# Autodesk Inventor assembly: Craftsman Socket U-Joint
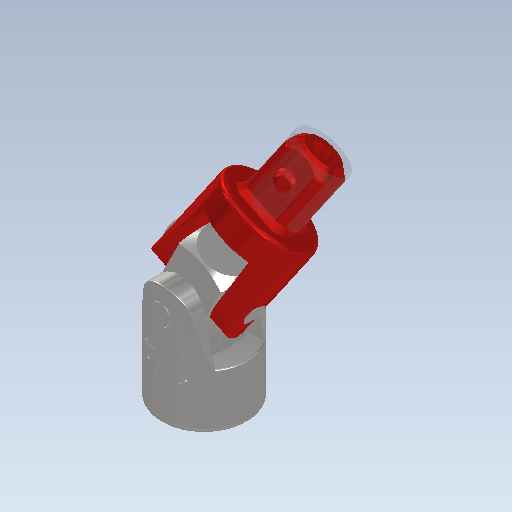
[picture p0: Inventor's stored thumbnail of the model, 512x512]
Saved by Autodesk Inventor 2020 (Build 240168000, 168)
## iProperties
Created: 2013-08-30
Part Number: Craftsman Socket U-Joint
Document SubType Name: Assembly
Designer: Vikki
Sending System: SolidWorks 2012
Last Author: MBryant
Last Saved: 2013-08-30
WEIGHT: 0.048
MX_MODIFIED: true
Author: Vikki
## Documents named in this file (4)
- D:\borewell rescuebot\pll manipulator files\sps manipulator\craftsman-3-pc-universal-joint-set-1.snapshot.1\Craftsman Socket U-Joint.iam
- D:\borewell rescuebot\pll manipulator files\sps manipulator\craftsman-3-pc-universal-joint-set-1.snapshot.1\Craftsman Socket U-Joint Base.ipt
- D:\borewell rescuebot\pll manipulator files\sps manipulator\craftsman-3-pc-universal-joint-set-1.snapshot.1\Craftsman Socket U-Joint Intermediate Body.ipt
- D:\borewell rescuebot\pll manipulator files\sps manipulator\craftsman-3-pc-universal-joint-set-1.snapshot.1\Craftsman Socket U-Joint Drive.ipt
## Components (3 placed, 3 different names)
1. Craftsman Socket U-Joint Base:1 — Mate:1, Mate:2
2. Craftsman Socket U-Joint Intermediate Body:1 — Mate:1, Mate:2, Mate:3, Mate:4
3. Craftsman Socket U-Joint Drive:1 — Mate:3, Mate:4
## Relationships (4: Mate 4)
- Mate:1: Craftsman Socket U-Joint Base:1 ↔ Craftsman Socket U-Joint Intermediate Body:1
- Mate:2: Craftsman Socket U-Joint Base:1 ↔ Craftsman Socket U-Joint Intermediate Body:1
- Mate:3: Craftsman Socket U-Joint Intermediate Body:1 ↔ Craftsman Socket U-Joint Drive:1
- Mate:4: Craftsman Socket U-Joint Intermediate Body:1 ↔ Craftsman Socket U-Joint Drive:1
